# Autodesk Inventor assembly: WOODLEG
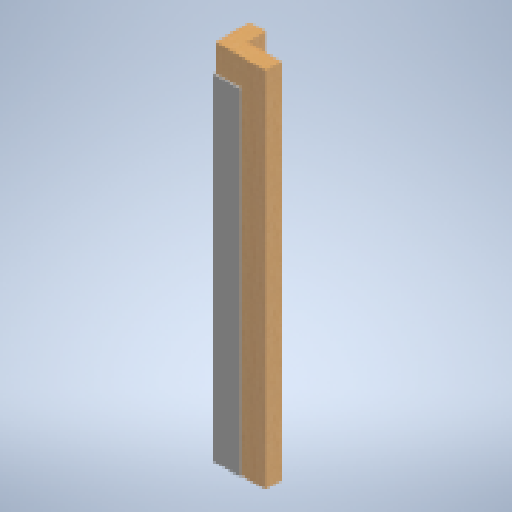
[picture p0: Inventor's stored thumbnail of the model, 512x512]
Saved by Autodesk Inventor 2023 (Build 270158000, 158)
## iProperties
Created: 2022-07-13
Part Number: WOODLEG
Document SubType Name: Assembly
Designer: plebbb
Author: plebbb
## Documents named in this file (3)
- D:\Users\plebbb\Desktop\CNC_Project\WOODLEG.iam
- D:\Users\plebbb\Desktop\CNC_Project\WOOD\2x4x40.ipt
- D:\Users\plebbb\Desktop\CNC_Project\L_Channel_SHORT.ipt
## Components (3 placed, 2 different names)
1. 2x4x40:1 — Mate:2, Mate:3, Flush:2
2. 2x4x40:2
3. L_Channel_SHORT:1 — Mate:2, Mate:3, Flush:2
## Relationships (5: Mate 3, Flush 2)
- [Mate]: 2x4x40:1 ↔ 2x4x40:2
- [Flush]: 2x4x40:1 ↔ 2x4x40:2
- Mate:2: 2x4x40:1 ↔ L_Channel_SHORT:1
- Mate:3: 2x4x40:1 ↔ L_Channel_SHORT:1
- Flush:2: 2x4x40:1 ↔ L_Channel_SHORT:1
